# Autodesk Inventor assembly: v1
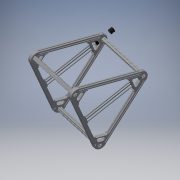
[picture p0: Inventor's stored thumbnail of the model, 180x180]
Saved by Autodesk Inventor 2019 (Build 230136000, 136)
## iProperties
Created: 2018-08-18
Part Number: v1
Document SubType Name: Assembly
Designer: Julia
Author: Julia
## Documents named in this file (7)
- C:\Users\Julia\Documents\Inventor\3D_Drucker_v01\v1.iam
- C:\Users\Julia\Documents\Inventor\3D_Drucker_v01\Rahmen.iam
- C:\Users\Julia\Documents\Inventor\3D_Drucker_v01\Rahmen_Y_Halterung_v1.ipt
- C:\Users\Julia\Documents\Inventor\3D_Drucker_v01\Y_Führungsstange.ipt
- C:\Users\Julia\Documents\Inventor\3D_Drucker_v01\Gewindestange_Y.ipt
- C:\Users\Julia\Downloads\stepper-motor-nema-17-with-timing-pulley-18-teeth-1.snapshot.2\MOTOR.ipt
- C:\Users\Julia\Downloads\M1173041- NEMA 17.ipt
## Components (11 placed, 6 different names)
1. Rahmen:1 [sub-assembly] — Mate:1, Angle:1, Mate:2, Mate:3, Mate:8, Angle:2, Mate:9, Mate:10
2. Rahmen_Y_Halterung_v1:1 — Mate:1, Angle:1, Mate:2, Mate:3, Mate:4, Mate:5, Mate:6, Mate:7, Mate:17, Mate:18
3. Y_Führungsstange:1 — Mate:4, Mate:5
4. Y_Führungsstange:2 — Mate:6, Mate:7
5. Y_Führungsstange:3 — Mate:12, Mate:14
6. Y_Führungsstange:4 — Mate:11, Mate:13
7. Rahmen_Y_Halterung_v1:2 — Mate:8, Angle:2, Mate:9, Mate:10, Mate:11, Mate:12, Mate:13, Mate:14, Mate:15, Mate:16
8. Gewindestange_Y:1 — Mate:17, Mate:18, Mate:19, Mate:20
9. Gewindestange_Y:2 — Mate:15, Mate:16
10. MOTOR:1 — Mate:19
11. M1173041- NEMA 17:1 — Mate:20
## Relationships (22: Mate 20, Angle 2)
- Mate:1: Rahmen:1 ↔ Rahmen_Y_Halterung_v1:1
- Angle:1 (0 deg): Rahmen:1 ↔ Rahmen_Y_Halterung_v1:1
- Mate:2: Rahmen:1 ↔ Rahmen_Y_Halterung_v1:1
- Mate:3: Rahmen:1 ↔ Rahmen_Y_Halterung_v1:1
- Mate:4: Rahmen_Y_Halterung_v1:1 ↔ Y_Führungsstange:1
- Mate:5: Rahmen_Y_Halterung_v1:1 ↔ Y_Führungsstange:1
- Mate:6: Rahmen_Y_Halterung_v1:1 ↔ Y_Führungsstange:2
- Mate:7: Rahmen_Y_Halterung_v1:1 ↔ Y_Führungsstange:2
- Mate:8: Rahmen:1 ↔ Rahmen_Y_Halterung_v1:2
- Angle:2 (0 deg): Rahmen:1 ↔ Rahmen_Y_Halterung_v1:2
- Mate:9: Rahmen:1 ↔ Rahmen_Y_Halterung_v1:2
- Mate:10: Rahmen:1 ↔ Rahmen_Y_Halterung_v1:2
- Mate:11: Y_Führungsstange:4 ↔ Rahmen_Y_Halterung_v1:2
- Mate:12: Y_Führungsstange:3 ↔ Rahmen_Y_Halterung_v1:2
- Mate:13: Y_Führungsstange:4 ↔ Rahmen_Y_Halterung_v1:2
- Mate:14: Y_Führungsstange:3 ↔ Rahmen_Y_Halterung_v1:2
- Mate:15: Rahmen_Y_Halterung_v1:2 ↔ Gewindestange_Y:2
- Mate:16: Rahmen_Y_Halterung_v1:2 ↔ Gewindestange_Y:2
- Mate:17: Rahmen_Y_Halterung_v1:1 ↔ Gewindestange_Y:1
- Mate:18: Rahmen_Y_Halterung_v1:1 ↔ Gewindestange_Y:1
- Mate:19: Gewindestange_Y:1 ↔ MOTOR:1
- Mate:20: Gewindestange_Y:1 ↔ M1173041- NEMA 17:1
